# Autodesk Inventor assembly: Full_assembly
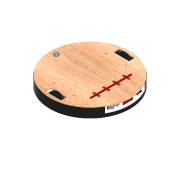
[picture p0: Inventor's stored thumbnail of the model, 180x180]
Saved by Autodesk Inventor 2020 (Build 240168000, 168)
## iProperties
Created: 2022-08-27
Part Number: Full_assembly
Document SubType Name: Assembly
Designer: Umair
Author: Umair
## Documents named in this file (3)
- C:\Users\pc\Dropbox\Umair\SCHOOL\1 Ma\Masterthesis\CAD\Full_assembly.iam
- C:\Users\pc\Dropbox\Umair\SCHOOL\1 Ma\Masterthesis\CAD\robot_top.iam
- C:\Users\pc\Dropbox\Umair\SCHOOL\1 Ma\Masterthesis\CAD\Robot_base.iam
## Components (2 placed, 2 different names)
1. robot_top:1 [sub-assembly] — Mate:1, Mate:2, Flush:1
2. Robot_base:1 [sub-assembly] — Mate:1, Mate:2, Flush:1
## Relationships (3: Mate 2, Flush 1)
- Mate:1 (100 mm): robot_top:1 ↔ Robot_base:1
- Mate:2: robot_top:1 ↔ Robot_base:1
- Flush:1: robot_top:1 ↔ Robot_base:1
